# Autodesk Inventor assembly: chaimber
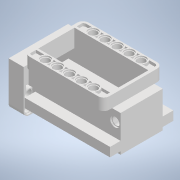
[picture p0: Inventor's stored thumbnail of the model, 180x180]
Saved by Autodesk Inventor 2021 (Build 250183000, 183)
## iProperties
Created: 2024-03-14
Part Number: chaimber
Document SubType Name: Assembly
Designer: 22hamfri
Author: 22hamfri
## Documents named in this file (5)
- C:\Users\22hamfri\Documents\School\Programmering\domino-bil\CAD\chaimber.iam
- C:\Users\22hamfri\Documents\School\Programmering\domino-bil\CAD\chaimber.ipt
- C:\Users\22hamfri\Documents\School\Programmering\domino-bil\CAD\chaimber-adapter.ipt
- C:\Users\22hamfri\Documents\School\Programmering\domino-bil\CAD\magazine-adapter.ipt
- C:\Users\22hamfri\Documents\School\Programmering\domino-bil\CAD\chaimber-bolt.ipt
## Components (4 placed, 4 different names)
1. chaimber:1 — Rigid:1, Rigid:2, Angle:1, Mate:1, bolt-action
2. chaimber-adapter:1 — Rigid:1
3. magazine-adapter:1 — Rigid:2
4. chaimber-bolt:1 — Angle:1, Mate:1, bolt-action
## Relationships (5: WeldJoint 2, Mate 2, Angle 1)
- Rigid:1 [WeldJoint]: chaimber:1 ↔ chaimber-adapter:1
- Rigid:2 [WeldJoint]: chaimber:1 ↔ magazine-adapter:1
- Angle:1 (180 deg): chaimber:1 ↔ chaimber-bolt:1
- Mate:1: chaimber:1 ↔ chaimber-bolt:1
- bolt-action [Mate]: chaimber:1 ↔ chaimber-bolt:1
